# Autodesk Inventor assembly: arm
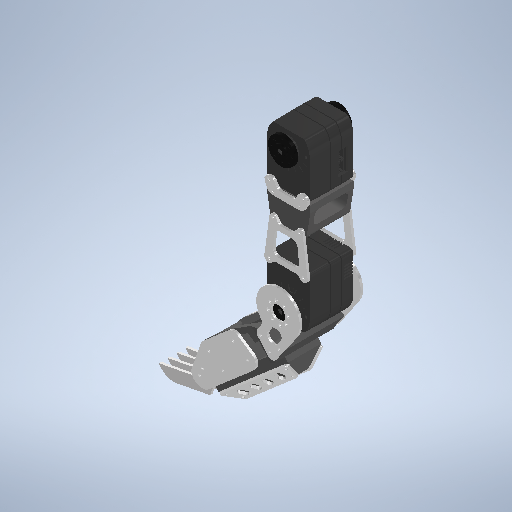
[picture p0: Inventor's stored thumbnail of the model, 512x512]
Saved by Autodesk Inventor 2026.1 (Build 301233020, 233B)
## iProperties
Created: 2024-10-12
Part Number: arm
Document SubType Name: Assembly
Designer: hibik
Author: hibik
## Documents named in this file (7)
- C:\Users\hibik\Documents\Robomech\HR\Eglantyne_mark2\hard\arm\arm.iam
- C:\Users\hibik\Documents\Robomech\HR\Eglantyne_mark2\hard\needed_model\KRS3300モータ.ipt
- C:\Users\hibik\Documents\Robomech\HR\Eglantyne_mark2\hard\needed_model\KRS3300サーボホーン.ipt
- C:\Users\hibik\Documents\Robomech\HR\Eglantyne_mark2\hard\arm\upper_arm.ipt
- C:\Users\hibik\Documents\Robomech\HR\Eglantyne_mark2\hard\arm\arm_middle.ipt
- C:\Users\hibik\Documents\Robomech\HR\Eglantyne_mark2\hard\arm\elbow.ipt
- C:\Users\hibik\Documents\Robomech\HR\Eglantyne_mark2\hard\arm_with_crow\hand.iam
## Components (12 placed, 6 different names)
1. KRS3300モータ:1 — 挿入:1, 挿入:2, 挿入:5, 挿入:6, 挿入:7, 挿入:8, メイト:2
2. KRS3300モータ:2 — 挿入:3, 挿入:4, 挿入:9, 挿入:10, 挿入:11, 挿入:12
3. KRS3300サーボホーン:1 — 挿入:1
4. KRS3300サーボホーン:2 — 挿入:2
5. KRS3300サーボホーン:3 — 挿入:3
6. KRS3300サーボホーン:4 — 挿入:4, 挿入:17
7. upper_arm:1 — 挿入:5, 挿入:6, メイト:3
8. upper_arm:2 — 挿入:7, 挿入:8, メイト:1
9. arm_middle:1 — メイト:1, メイト:2, メイト:3, 挿入:16, 角度:1
10. elbow:1 — 挿入:9, 挿入:12, 挿入:16, 角度:1
11. elbow:2 — 挿入:10, 挿入:11
12. hand:1 [sub-assembly] — 挿入:17
## Relationships (18: Insert 14, Mate 3, Angle 1)
- 挿入:1 [Insert]: KRS3300モータ:1 ↔ KRS3300サーボホーン:1
- 挿入:2 [Insert]: KRS3300モータ:1 ↔ KRS3300サーボホーン:2
- 挿入:3 [Insert]: KRS3300モータ:2 ↔ KRS3300サーボホーン:3
- 挿入:4 [Insert]: KRS3300モータ:2 ↔ KRS3300サーボホーン:4
- 挿入:5 [Insert]: KRS3300モータ:1 ↔ upper_arm:1
- 挿入:6 [Insert]: KRS3300モータ:1 ↔ upper_arm:1
- 挿入:7 [Insert]: KRS3300モータ:1 ↔ upper_arm:2
- 挿入:8 [Insert]: KRS3300モータ:1 ↔ upper_arm:2
- メイト:1 [Mate]: upper_arm:2 ↔ arm_middle:1
- メイト:2 [Mate] (1 mm): KRS3300モータ:1 ↔ arm_middle:1
- メイト:3 [Mate] (-3 mm): upper_arm:1 ↔ arm_middle:1
- 挿入:9 [Insert]: KRS3300モータ:2 ↔ elbow:1
- 挿入:10 [Insert]: KRS3300モータ:2 ↔ elbow:2
- 挿入:11 [Insert]: KRS3300モータ:2 ↔ elbow:2
- 挿入:12 [Insert]: KRS3300モータ:2 ↔ elbow:1
- 挿入:16 [Insert]: arm_middle:1 ↔ elbow:1
- 角度:1 [Angle] (0 deg): arm_middle:1 ↔ elbow:1
- 挿入:17 [Insert]: KRS3300サーボホーン:4 ↔ hand:1
